# Autodesk Inventor assembly: Wing nubs assembly
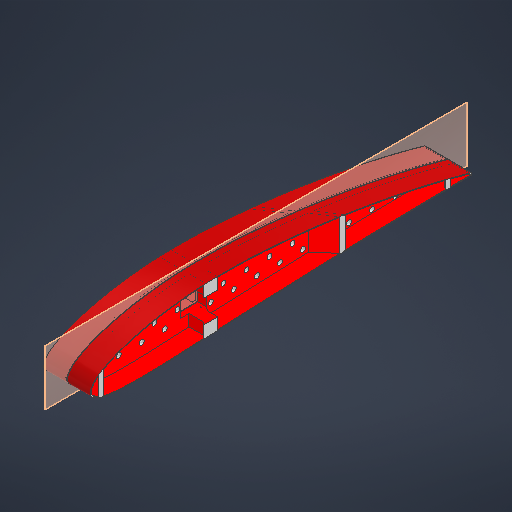
[picture p0: Inventor's stored thumbnail of the model, 512x512]
Saved by Autodesk Inventor 2026.1 (Build 301233000, 233)
## iProperties
Created: 2025-10-08
Part Number: Wing nubs assembly
Document SubType Name: Assembly
Designer: mateo
Author: mateo
## Documents named in this file (3)
- C:\GitHub\SWIFT-UAV\System_development\Pelican\CAD_model\v0.2.3\Parts\WingParts\Wing nubs assembly.iam
- C:\GitHub\SWIFT-UAV\System_development\Pelican\CAD_model\v0.2.3\Parts\WingParts\Wing Section - inset.ipt
- C:\GitHub\SWIFT-UAV\System_development\Pelican\CAD_model\v0.2.3\Parts\WingParts\Wing Section - inset hole.ipt
## Components (2 placed, 2 different names)
1. Wing Section - inset:1 — Insert:1
2. Wing Section - inset hole:1 — Insert:1
## Relationships (1: Insert 1)
- Insert:1 (-2.54 mm): Wing Section - inset:1 ↔ Wing Section - inset hole:1
